# Autodesk Inventor assembly: COTS_WCP_Full_Kraken
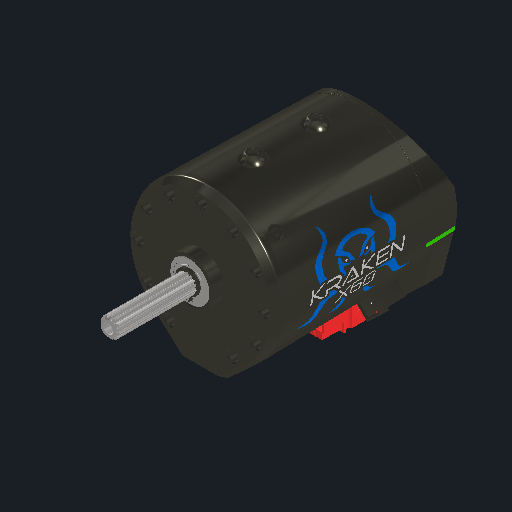
[picture p0: Inventor's stored thumbnail of the model, 512x512]
Saved by Autodesk Inventor 2024 (Build 280153000, 153)
## iProperties
Created: 2024-01-04
Part Number: COTS_WCP_Full_Kraken
Document SubType Name: Assembly
Designer: Marshall
Author: Marshall
## Documents named in this file (3)
- C:\Users\Marshall\Documents\CacheCAD\Crescendo Robot 2\COTS Library\Motors\COTS_WCP_Full_Kraken.iam
- C:\Users\Marshall\Documents\CacheCAD\Crescendo Robot 2\COTS Library\Motors\COTS_WCP-0940_Kraken_No_Powerpole.ipt
- C:\Users\Marshall\Documents\CacheCAD\Crescendo Robot 2\COTS Library\Motors\COTS_WCP-1380_Kraken_Powerpole.ipt
## Components (2 placed, 2 different names)
1. COTS_WCP-0940_Kraken_No_Powerpole:1 — Mate:1, Flush:1, Flush:2, Flush:3, Mate:2, Mate:3
2. COTS_WCP-1380_Kraken_Powerpole:1 — Mate:1, Mate:2, Mate:3
## Relationships (6: Mate 3, Flush 3)
- Mate:1: COTS_WCP-0940_Kraken_No_Powerpole:1 ↔ COTS_WCP-1380_Kraken_Powerpole:1
- Flush:1: COTS_WCP-0940_Kraken_No_Powerpole:1
- Flush:2: COTS_WCP-0940_Kraken_No_Powerpole:1
- Flush:3: COTS_WCP-0940_Kraken_No_Powerpole:1
- Mate:2: COTS_WCP-0940_Kraken_No_Powerpole:1 ↔ COTS_WCP-1380_Kraken_Powerpole:1
- Mate:3: COTS_WCP-0940_Kraken_No_Powerpole:1 ↔ COTS_WCP-1380_Kraken_Powerpole:1
